# Autodesk Inventor assembly: forgoresz
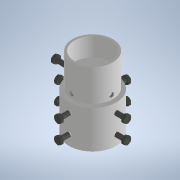
[picture p0: Inventor's stored thumbnail of the model, 180x180]
Saved by Autodesk Inventor 2021.4 (Build 254397000, 397)
## iProperties
Created: 2023-12-02
Part Number: forgoresz
Document SubType Name: Assembly
Designer: vtoth
Author: vtoth
## Documents named in this file (5)
- C:\Users\vtoth\OneDrive - Budapesti Műszaki és Gazdaságtudományi Egyetem\5_felev\CAD\hf2_v2\forgoresz.iam
- C:\Users\vtoth\OneDrive - Budapesti Műszaki és Gazdaságtudományi Egyetem\5_felev\CAD\hf2_v2\forgo_also.ipt
- C:\Users\vtoth\OneDrive - Budapesti Műszaki és Gazdaságtudományi Egyetem\5_felev\CAD\hf2_v2\forgo_felso.ipt
- C:\Users\vtoth\OneDrive - Budapesti Műszaki és Gazdaságtudományi Egyetem\5_felev\CAD\hf2_v2\ContentCenter\en-US\ISO 4018\ISO 4018 - M8 x 16.ipt
- C:\Users\vtoth\OneDrive - Budapesti Műszaki és Gazdaságtudományi Egyetem\5_felev\CAD\hf2_v2\ContentCenter\en-US\ISO 4018\ISO 4018 - M8 x 40.ipt
## Components (11 placed, 4 different names)
1. forgo_also:1 — Mate:2, Mate:3, Mate:5, Tangent:1, Insert:1
2. forgo_felso:1 — Mate:4, Insert:1, Mate:8
3. ISO 4018 M8 x 40:1 — Mate:4, Tangent:1, Mate:8
4. ISO 4018 M8 x 16:2 — Mate:2, Angle:3, Flush:3, Mate:5
5. ISO 4018 M8 x 16:3 — Mate:3, Angle:3, Flush:3
6. ISO 4018 M8 x 16:4
7. ISO 4018 M8 x 16:5
8. ISO 4018 M8 x 16:6
9. ISO 4018 M8 x 16:7
10. ISO 4018 M8 x 16:8
11. ISO 4018 M8 x 16:9
## Component patterns: (4 elements, first: ISO 4018 M8 x 16:2 + ISO 4018 M8 x 16:3)
## Relationships (9: Mate 5, Angle 1, Flush 1, Tangent 1, Insert 1)
- Mate:2: forgo_also:1 ↔ ISO 4018 M8 x 16:2
- Mate:3: forgo_also:1 ↔ ISO 4018 M8 x 16:3
- Angle:3 (0 deg): ISO 4018 M8 x 16:2 ↔ ISO 4018 M8 x 16:3
- Flush:3: ISO 4018 M8 x 16:2 ↔ ISO 4018 M8 x 16:3
- Mate:4: forgo_felso:1 ↔ ISO 4018 M8 x 40:1
- Mate:5: forgo_also:1 ↔ ISO 4018 M8 x 16:2
- Tangent:1: forgo_also:1 ↔ ISO 4018 M8 x 40:1
- Insert:1: forgo_also:1 ↔ forgo_felso:1
- Mate:8: forgo_felso:1 ↔ ISO 4018 M8 x 40:1
